# Autodesk Inventor assembly: left_grabber
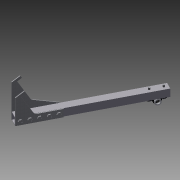
[picture p0: Inventor's stored thumbnail of the model, 180x180]
Saved by Autodesk Inventor 2011 (Build 150239000, 239)
## iProperties
Created: 2013-01-18
Part Number: left_grabber
Document SubType Name: Assembly
Designer: Christopher
Author: Christopher
## Documents named in this file (8)
- F:\Users\Christopher\Documents\GitHub\2013CAD\2013 robot\forklift\Pneumatics and frame grabbers\left_grabber.iam
- F:\Users\Christopher\Documents\GitHub\2013CAD\2013 robot\forklift\Pneumatics and frame grabbers\1tube_10_framegrabberarm.ipt
- F:\Users\Christopher\Documents\GitHub\2013CAD\2013 robot\forklift\Pneumatics and frame grabbers\grabber_plate_metal_hook.ipt
- F:\Users\Christopher\Documents\GitHub\2013CAD\2013 robot\forklift\Pneumatics and frame grabbers\grabber_plate_metal_hook_long.ipt
- F:\Users\Christopher\Documents\GitHub\2013CAD\2013 robot\forklift\Misc parts\1.5_bolt_.25_20.ipt
- F:\Users\Christopher\Documents\GitHub\2013CAD\2013 robot\forklift\Misc parts\nut_.25_20.ipt
- F:\Users\Christopher\Documents\GitHub\2013CAD\2013 robot\forklift\Misc parts\.5inch_side_bearing.ipt
- F:\Users\Christopher\Documents\GitHub\2013CAD\2013 robot\forklift\Misc parts\.5_inch_axle_bushing.ipt
## Components (18 placed, 7 different names)
1. 1tube_10_framegrabberarm:1 — Insert:23, Insert:24, Insert:25, Insert:26, Insert:37, Insert:38
2. grabber_plate_metal_hook:1 — Insert:25, Insert:26, Insert:27, Insert:28, Insert:29, Insert:30, Insert:31
3. grabber_plate_metal_hook_long:1 — Insert:23, Insert:24, Insert:32, Insert:33, Insert:34, Insert:35, Insert:36
4. 1.5_bolt_.25_20:6 — Insert:20
5. 1.5_bolt_.25_20:7 — Insert:19
6. .5inch_side_bearing:1 — Insert:17, Insert:18, Insert:19, Insert:20, Insert:37, Insert:38
7. .5_inch_axle_bushing:1 — Insert:17
8. .5_inch_axle_bushing:2 — Insert:18
9. 1.5_bolt_.25_20:8 — Insert:27
10. 1.5_bolt_.25_20:9 — Insert:28
11. 1.5_bolt_.25_20:10 — Insert:29
12. 1.5_bolt_.25_20:11 — Insert:30
13. 1.5_bolt_.25_20:12 — Insert:31
14. nut_.25_20:8 — Insert:35
15. nut_.25_20:9 — Insert:34
16. nut_.25_20:10 — Insert:33
17. nut_.25_20:11 — Insert:32
18. nut_.25_20:12 — Insert:36
## Relationships (20: Insert 20)
- Insert:17: .5inch_side_bearing:1 ↔ .5_inch_axle_bushing:1
- Insert:18: .5inch_side_bearing:1 ↔ .5_inch_axle_bushing:2
- Insert:19: 1.5_bolt_.25_20:7 ↔ .5inch_side_bearing:1
- Insert:20: 1.5_bolt_.25_20:6 ↔ .5inch_side_bearing:1
- Insert:23: 1tube_10_framegrabberarm:1 ↔ grabber_plate_metal_hook_long:1
- Insert:24: 1tube_10_framegrabberarm:1 ↔ grabber_plate_metal_hook_long:1
- Insert:25: 1tube_10_framegrabberarm:1 ↔ grabber_plate_metal_hook:1
- Insert:26: 1tube_10_framegrabberarm:1 ↔ grabber_plate_metal_hook:1
- Insert:27: grabber_plate_metal_hook:1 ↔ 1.5_bolt_.25_20:8
- Insert:28: grabber_plate_metal_hook:1 ↔ 1.5_bolt_.25_20:9
- Insert:29: grabber_plate_metal_hook:1 ↔ 1.5_bolt_.25_20:10
- Insert:30: grabber_plate_metal_hook:1 ↔ 1.5_bolt_.25_20:11
- Insert:31: grabber_plate_metal_hook:1 ↔ 1.5_bolt_.25_20:12
- Insert:32: grabber_plate_metal_hook_long:1 ↔ nut_.25_20:11
- Insert:33: grabber_plate_metal_hook_long:1 ↔ nut_.25_20:10
- Insert:34: grabber_plate_metal_hook_long:1 ↔ nut_.25_20:9
- Insert:35: grabber_plate_metal_hook_long:1 ↔ nut_.25_20:8
- Insert:36: grabber_plate_metal_hook_long:1 ↔ nut_.25_20:12
- Insert:37: 1tube_10_framegrabberarm:1 ↔ .5inch_side_bearing:1
- Insert:38: 1tube_10_framegrabberarm:1 ↔ .5inch_side_bearing:1
